# Autodesk Inventor assembly: Ensamblaje
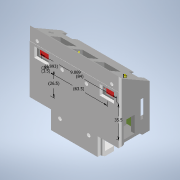
[picture p0: Inventor's stored thumbnail of the model, 180x180]
Saved by Autodesk Inventor 2021 (Build 250183000, 183)
## iProperties
Created: 2021-10-29
Part Number: Ensamblaje
Document SubType Name: Weldment
Designer: Juan Camilo
Weld Material: Welded Aluminum-6061
Author: Juan Camilo
## Documents named in this file (11)
- C:\Users\Juan Camilo\OneDrive - Universidad de los Andes\Escritorio\Onixium\Ensamblaje.iam
- C:\Users\Juan Camilo\OneDrive - Universidad de los Andes\Escritorio\Onixium\Base Onixium.ipt
- C:\Users\Juan Camilo\OneDrive - Universidad de los Andes\Escritorio\Onixium\Batería.ipt
- C:\Users\Juan Camilo\OneDrive - Universidad de los Andes\Escritorio\Onixium\Cuchilla Versión 1.ipt
- C:\Users\Juan Camilo\OneDrive - Universidad de los Andes\Escritorio\Onixium\PlacaInferior.ipt
- C:\Users\Juan Camilo\OneDrive - Universidad de los Andes\Escritorio\Onixium\PosiblePlaca.ipt
- C:\Users\Juan Camilo\OneDrive - Universidad de los Andes\Escritorio\Onixium\Puente H.ipt
- C:\Users\Juan Camilo\OneDrive - Universidad de los Andes\Escritorio\Onixium\Arduino Nano.ipt
- C:\Users\Juan Camilo\OneDrive - Universidad de los Andes\Escritorio\Onixium\PiezaAtras.ipt
- C:\Users\Juan Camilo\OneDrive - Universidad de los Andes\Escritorio\Onixium\SensorDeLinea.ipt
- C:\Users\Juan Camilo\OneDrive - Universidad de los Andes\Escritorio\Onixium\TapaOnixium.ipt
## Components (11 placed, 10 different names)
1. Base Onixium:1 — Coincidencia:1, Coincidencia:2, Coincidencia:3, Coincidencia:4, Coincidencia:8, Coincidencia:13, Coincidencia:14, Coincidencia:15, Rígido:2
2. Batería:1 — Coincidencia:1, Coincidencia:2, Coincidencia:3
3. Cuchilla Versión 1:1 — Coincidencia:4, Rígido:1
4. PosiblePlaca:1 — Coincidencia:8, Coincidencia:9, Coincidencia:10
5. Puente H:1 — Coincidencia:9
6. Arduino Nano:1 — Coincidencia:10
7. PlacaInferior:1 — Rígido:1
8. PiezaAtras:1 — Coincidencia:13
9. SensorDeLinea:1 — Coincidencia:15
10. SensorDeLinea:2 — Coincidencia:14
11. TapaOnixium:1 — Rígido:2
## Relationships (12: Mate 10, WeldJoint 2)
- Coincidencia:1 [Mate]: Base Onixium:1 ↔ Batería:1
- Coincidencia:2 [Mate] (3 mm): Base Onixium:1 ↔ Batería:1
- Coincidencia:3 [Mate] (15.5 mm): Base Onixium:1 ↔ Batería:1
- Coincidencia:4 [Mate]: Base Onixium:1 ↔ Cuchilla Versión 1:1
- Coincidencia:8 [Mate]: Base Onixium:1 ↔ PosiblePlaca:1
- Coincidencia:9 [Mate]: PosiblePlaca:1 ↔ Puente H:1
- Coincidencia:10 [Mate]: PosiblePlaca:1 ↔ Arduino Nano:1
- Rígido:1 [WeldJoint]: Cuchilla Versión 1:1 ↔ PlacaInferior:1
- Coincidencia:13 [Mate]: Base Onixium:1 ↔ PiezaAtras:1
- Coincidencia:14 [Mate]: Base Onixium:1 ↔ SensorDeLinea:2
- Coincidencia:15 [Mate]: Base Onixium:1 ↔ SensorDeLinea:1
- Rígido:2 [WeldJoint]: Base Onixium:1 ↔ TapaOnixium:1
